# Autodesk Inventor assembly: Mecanum assembly Right
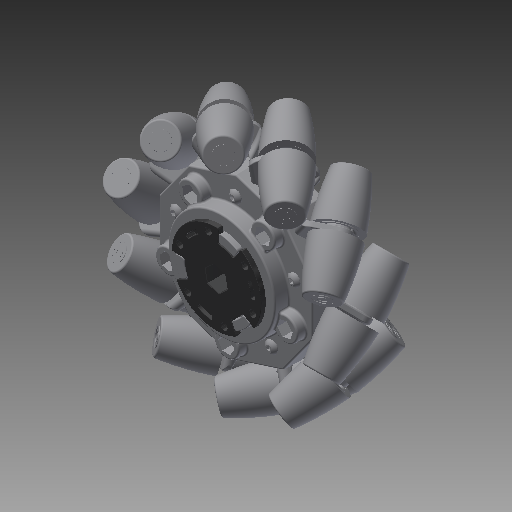
[picture p0: Inventor's stored thumbnail of the model, 512x512]
Saved by Autodesk Inventor 2018 (Build 220112000, 112)
## iProperties
Created: 2019-01-19
Part Number: Mecanum assembly Right
Document SubType Name: Assembly
Designer: maste
Author: maste
## Documents named in this file (4)
- C:\Users\s-2512711\Desktop\Github\2019CAD\Drivebase but Calvin is a mad man\Mecanum assembly Right.iam
- C:\Users\s-2512711\Desktop\Github\2019CAD\Outdated Project Folders\Summer Drivebase\1_2_Hex_Bore_Plastic_VersaHub_217-4009.ipt
- C:\Users\s-2512711\Desktop\Github\2019CAD\Outdated Project Folders\Summer Drivebase\1_2_Hex_Bore_Aluminum_VersaHub_217-2592.ipt
- C:\Users\s-2512711\Desktop\Github\2019CAD\Drivebase but Calvin is a mad man\6_Mecanum_Wheel_Right_217-2586.ipt
## Components (3 placed, 3 different names)
1. 1_2_Hex_Bore_Plastic_VersaHub_217-4009:1 — Mate:1, Mate:2, Mate:3
2. 1_2_Hex_Bore_Aluminum_VersaHub_217-2592:1 — Mate:4, Mate:5, Mate:6
3. 6_Mecanum_Wheel_Right_217-2586:1 — Mate:1, Mate:2, Mate:3, Mate:4, Mate:5, Mate:6
## Relationships (6: Mate 6)
- Mate:1: 1_2_Hex_Bore_Plastic_VersaHub_217-4009:1 ↔ 6_Mecanum_Wheel_Right_217-2586:1
- Mate:2: 1_2_Hex_Bore_Plastic_VersaHub_217-4009:1 ↔ 6_Mecanum_Wheel_Right_217-2586:1
- Mate:3: 1_2_Hex_Bore_Plastic_VersaHub_217-4009:1 ↔ 6_Mecanum_Wheel_Right_217-2586:1
- Mate:4: 1_2_Hex_Bore_Aluminum_VersaHub_217-2592:1 ↔ 6_Mecanum_Wheel_Right_217-2586:1
- Mate:5: 1_2_Hex_Bore_Aluminum_VersaHub_217-2592:1 ↔ 6_Mecanum_Wheel_Right_217-2586:1
- Mate:6: 1_2_Hex_Bore_Aluminum_VersaHub_217-2592:1 ↔ 6_Mecanum_Wheel_Right_217-2586:1
